# Autodesk Inventor assembly: 90-10-0114
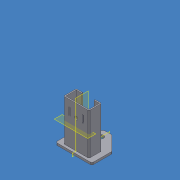
[picture p0: Inventor's stored thumbnail of the model, 180x180]
Saved by Autodesk Inventor 2015 SP1 (Build 190203100, 203)
## iProperties
Created: 2007-07-04
Part Number: 90-10-0114
Document SubType Name: Assembly
Designer: kurt
Manufacturer: Standard
Standards Organization: Custom
Author: kurt
## Documents named in this file (3)
- F:\Tekeningen\bibliotheek\poten\Sub-assemblys\90-10-0114.iam
- F:\Tekeningen\bibliotheek\poten\onderdelen\90-05-0114.ipt
- F:\Tekeningen\bibliotheek\poten\onderdelen\90-01-0000.ipt
## Components (2 placed, 2 different names)
1. 90-05-0114:1 — Mate:3, Mate:4, Flush:2
2. 90-01-0000:1 — Mate:1, Mate:2, Flush:1, Mate:3, Mate:4, Flush:2
## Relationships (6: Mate 4, Flush 2)
- Mate:1: 90-01-0000:1
- Mate:2: 90-01-0000:1
- Flush:1: 90-01-0000:1
- Mate:3: 90-05-0114:1 ↔ 90-01-0000:1
- Mate:4: 90-05-0114:1 ↔ 90-01-0000:1
- Flush:2: 90-05-0114:1 ↔ 90-01-0000:1
